# Autodesk Inventor assembly: Assembly rangka
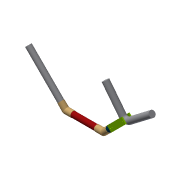
[picture p0: Inventor's stored thumbnail of the model, 180x180]
Saved by Autodesk Inventor 2018 (Build 220112000, 112)
## iProperties
Created: 2019-12-18
Part Number: Assembly rangka
Document SubType Name: Assembly
Designer: Ibnu
Author: Ibnu
## Documents named in this file (8)
- C:\Users\Ibnu\Documents\Inventor\ROCKER BOGIE ROBOT\Assembly rangka.iam
- C:\Users\Ibnu\Documents\Inventor\ROCKER BOGIE ROBOT\17cm.ipt
- C:\Users\Ibnu\Documents\Inventor\ROCKER BOGIE ROBOT\knee 45.ipt
- C:\Users\Ibnu\Documents\Inventor\ROCKER BOGIE ROBOT\8,5cm.ipt
- C:\Users\Ibnu\Documents\Inventor\ROCKER BOGIE ROBOT\8,5 hub.ipt
- C:\Users\Ibnu\Documents\Inventor\ROCKER BOGIE ROBOT\plat.ipt
- C:\Users\Ibnu\Documents\Inventor\ROCKER BOGIE ROBOT\25cm.ipt
- C:\Users\Ibnu\Documents\Inventor\ROCKER BOGIE ROBOT\L90roda.ipt
## Components (9 placed, 7 different names)
1. 17cm:1 — Rigid:3, Rigid:4
2. knee 45:1 — Rigid:4, Insert:1
3. knee 45:2 — Rigid:3, Rotational:1
4. 8,5cm:2 — Rigid:1, Insert:1
5. 8,5 hub:2 — Rigid:1, Mate:1, Mate:2, Tangent:1, Angle:1, Mate:3, Mate:4
6. plat:1 — Mate:1, Mate:2, Tangent:1, Angle:1, Flush:1, Mate:6
7. 25cm:1 — Rotational:1
8. plat:2 — Mate:3, Mate:4, Flush:1, Mate:5, Tangent:2
9. L90roda:1 — Mate:5, Mate:6, Tangent:2
## Relationships (15: Mate 6, WeldJoint 3, Tangent 2, Angle 1, RevoluteJoint 1, Flush 1, Insert 1)
- Rigid:1 [WeldJoint]: 8,5cm:2 ↔ 8,5 hub:2
- Rigid:3 [WeldJoint] (-28 mm): 17cm:1 ↔ knee 45:2
- Rigid:4 [WeldJoint] (-28 mm): 17cm:1 ↔ knee 45:1
- Mate:1: 8,5 hub:2 ↔ plat:1
- Mate:2: 8,5 hub:2 ↔ plat:1
- Tangent:1: 8,5 hub:2 ↔ plat:1
- Angle:1 (0 deg): 8,5 hub:2 ↔ plat:1
- Rotational:1 [RevoluteJoint] (-28 mm): knee 45:2 ↔ 25cm:1
- Mate:3: 8,5 hub:2 ↔ plat:2
- Mate:4: 8,5 hub:2 ↔ plat:2
- Flush:1 (-34 mm): plat:1 ↔ plat:2
- Insert:1 (-28 mm): knee 45:1 ↔ 8,5cm:2
- Mate:5: plat:2 ↔ L90roda:1
- Mate:6: plat:1 ↔ L90roda:1
- Tangent:2: plat:2 ↔ L90roda:1
